# Autodesk Inventor assembly: Assembly1
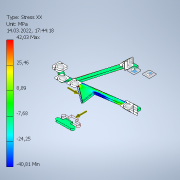
[picture p0: Inventor's stored thumbnail of the model, 180x180]
Saved by Autodesk Inventor 2022 (Build 260153000, 153)
## iProperties
Created: 2022-03-14
Part Number: Assembly1
Document SubType Name: Assembly
Designer: br4ch
Author: br4ch
## Documents named in this file (21)
- C:\Users\br4ch\M-and-Ms\Final exam\Assembly1.iam
- C:\Users\br4ch\M-and-Ms\Final exam\Part1.ipt
- C:\Users\br4ch\M-and-Ms\Final exam\Part3.ipt
- C:\Users\br4ch\M-and-Ms\Final exam\Part2.ipt
- C:\Users\br4ch\M-and-Ms\Final exam\Slider1.ipt
- C:\Users\br4ch\M-and-Ms\Final exam\Slider2.ipt
- C:\Users\br4ch\M-and-Ms\Final exam\PartRef.ipt
- C:\Users\br4ch\M-and-Ms\Final exam\slot1.ipt
- C:\Users\br4ch\M-and-Ms\Final exam\axis1.ipt
- C:\Users\br4ch\M-and-Ms\Final exam\Assembly1\AIP\FEA\dwrlbm10g.fins
- C:\Users\br4ch\M-and-Ms\Final exam\Assembly1\AIP\FEA\dwrlbm11c.fsat
- C:\Users\br4ch\M-and-Ms\Final exam\Assembly1\AIP\FEA\dwrlbm11c.ftes
- C:\Users\br4ch\M-and-Ms\Final exam\Assembly1\AIP\FEA\dwrlbm11c.fwiz
- C:\Users\br4ch\M-and-Ms\Final exam\Assembly1\AIP\FEA\dwrlbm15s.fmsh
- C:\Users\br4ch\M-and-Ms\Final exam\Assembly1\AIP\FEA\dwrlbm15t.fres
- C:\Users\br4ch\M-and-Ms\Final exam\Assembly1\AIP\FEA\dwronem80.fins
- C:\Users\br4ch\M-and-Ms\Final exam\Assembly1\AIP\FEA\dwronem80.fsat
- C:\Users\br4ch\M-and-Ms\Final exam\Assembly1\AIP\FEA\dwronem80.ftes
- C:\Users\br4ch\M-and-Ms\Final exam\Assembly1\AIP\FEA\dwronem80.fwiz
- C:\Users\br4ch\M-and-Ms\Final exam\Assembly1\AIP\FEA\dwronemcg.fmsh
- C:\Users\br4ch\M-and-Ms\Final exam\Assembly1\AIP\FEA\dwronemch.fres
## Components (9 placed, 8 different names)
1. Part1:1 — Rotational:1, Mate:1, Symmetry:1, Angle:1, Rotational:5
2. Part3:1 — Rotational:7, Rotational:6
3. Part2:1 — Rotational:1, Rotational:4, Symmetry:1, Angle:3, Rotational:6
4. Slider1:1 — Rotational:7, Flush:8, Mate:9
5. Slider2:1 — Rotational:4, Angle:5, Mate:6, Flush:7
6. PartRef:1 — Angle:1, Angle:3, Angle:4, Angle:5
7. slot1:1 — Mate:8, Flush:8, Mate:9
8. axis1:1 — Rotational:5, Angle:4, Flush:1, Mate:7
9. slot1:2 — Mate:6, Flush:7, Mate:7
## Relationships (21: Mate 7, RevoluteJoint 5, Angle 4, Flush 4, Symmetry 1)
- Rotational:1 [RevoluteJoint]: Part1:1 ↔ Part2:1
- Rotational:4 [RevoluteJoint]: Part2:1 ↔ Slider2:1
- Mate:1: Part1:1
- Symmetry:1: Part1:1 ↔ Part2:1
- Mate:2
- Mate:3
- Angle:1 (0 deg): Part1:1 ↔ PartRef:1
- Angle:3 (0 deg): Part2:1 ↔ PartRef:1
- Rotational:5 [RevoluteJoint]: Part1:1 ↔ axis1:1
- Angle:4 (0 deg): PartRef:1 ↔ axis1:1
- Flush:1 (-5 mm): axis1:1
- Flush:2 (100 mm)
- Angle:5 (0 deg): Slider2:1 ↔ PartRef:1
- Mate:6: Slider2:1 ↔ slot1:2
- Flush:7: Slider2:1 ↔ slot1:2
- Mate:7: axis1:1 ↔ slot1:2
- Rotational:7 [RevoluteJoint]: Part3:1 ↔ Slider1:1
- Rotational:6 [RevoluteJoint]: Part3:1 ↔ Part2:1
- Mate:8: slot1:1
- Flush:8: Slider1:1 ↔ slot1:1
- Mate:9: Slider1:1 ↔ slot1:1
## Named parameters: sa_0 = 50000, sa_1 = 0, sa_2 = 0, sa_3 = 981, sa_4 = 1000, sa_5 = 0, sa_6 = 0, sa_7 = 981
note: some values were not read from the file. Shown as the stored number, unit unknown: "sa_0", "sa_1", "sa_2", "sa_3", "sa_4", "sa_5", "sa_6", "sa_7".
